# Autodesk Inventor assembly: r_wheel_assembly
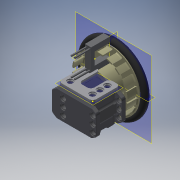
[picture p0: Inventor's stored thumbnail of the model, 180x180]
Saved by Autodesk Inventor 2016 (Build 200138000, 138)
## iProperties
Created: 2016-02-15
Part Number: r_wheel_assembly
Document SubType Name: Assembly
Designer: jforce
Author: jforce
## Documents named in this file (6)
- C:\Users\jforce\Dropbox\gmu\ece590 (Selective Sync Conflict)\models3\r_wheel_assembly.iam
- C:\Users\jforce\Dropbox\gmu\ece590 (Selective Sync Conflict)\models3\p_inter.ipt
- C:\Users\jforce\Dropbox\gmu\ece590 (Selective Sync Conflict)\models3\tire.ipt
- C:\Users\jforce\Dropbox\gmu\ece590 (Selective Sync Conflict)\models3\wheel.ipt
- C:\Users\jforce\Dropbox\gmu\ece590 (Selective Sync Conflict)\models3\XL-320_servo.ipt
- C:\Users\jforce\Dropbox\gmu\ece590 (Selective Sync Conflict)\models3\p_int_mount.ipt
## Components (5 placed, 5 different names)
1. p_inter:1 — Mate:8, Mate:9
2. tire:1 — Mate:3, Mate:4
3. wheel:1 — Mate:1, Mate:2
4. XL-320_servo:1 — Mate:1, Mate:2, Angle:1, Mate:5, Mate:6, Mate:7
5. p_int_mount:1 — Mate:5, Mate:6, Mate:7, Mate:8, Mate:9
## Relationships (10: Mate 9, Angle 1)
- Mate:1: wheel:1 ↔ XL-320_servo:1
- Mate:2: wheel:1 ↔ XL-320_servo:1
- Angle:1 (0 deg): XL-320_servo:1
- Mate:3: tire:1
- Mate:4: tire:1
- Mate:5: XL-320_servo:1 ↔ p_int_mount:1
- Mate:6: XL-320_servo:1 ↔ p_int_mount:1
- Mate:7: XL-320_servo:1 ↔ p_int_mount:1
- Mate:8: p_inter:1 ↔ p_int_mount:1
- Mate:9: p_inter:1 ↔ p_int_mount:1
